# Autodesk Inventor assembly: 足裏_1_1
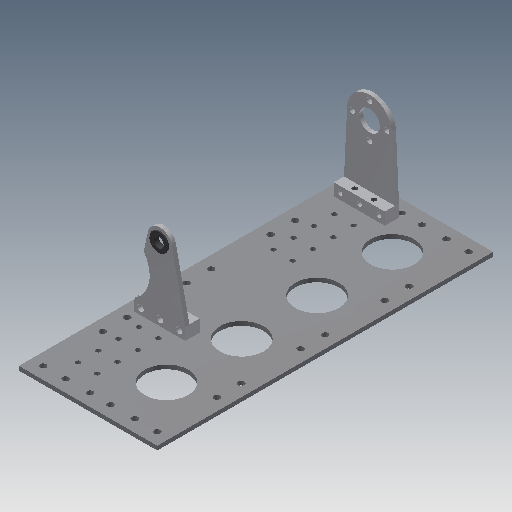
[picture p0: Inventor's stored thumbnail of the model, 512x512]
Saved by Autodesk Inventor 2017.3 (Build 213256000, 256)
## iProperties
Created: 2016-05-01
Part Number: 足裏_1_1
Document SubType Name: Assembly
Designer: hiroaki
Mass: 45.3916 g
Surface Area: 270.384 cm^2
Volume: 23.3732 cm^3
Density: 1.94204 g/cm^3
Author: hiroaki
## Documents named in this file (6)
- C:\Users\haya\Desktop\GankenKun0_5\下半身\足裏\足裏_1_1.iam
- C:\Users\haya\Desktop\GankenKun0_5\下半身\足裏\足裏_メインフレーム_1_1.ipt
- C:\Users\haya\Desktop\GankenKun0_5\下半身\足裏\足裏_メインフレーム_1_2.ipt
- C:\Users\haya\Desktop\GankenKun0_5\下半身\足裏\足裏_サブフレーム_1_1.ipt
- C:\Users\haya\Desktop\GankenKun0_5\既製品\NSK_RB_MF85ZZ\MF85ZZ.iam
- C:\Users\haya\Desktop\GankenKun0_5\下半身\足裏\足裏_メインフレーム_1_3.ipt
## Components (6 placed, 5 different names)
1. 足裏_メインフレーム_1_1:1 — メイト:1, フラッシュ:1, フラッシュ:2, メイト:2, フラッシュ:3, メイト:3, 挿入:4, 挿入:5, 挿入:6
2. 足裏_メインフレーム_1_2:1 — メイト:2, フラッシュ:3, メイト:3, 挿入:1, 挿入:2, 挿入:3, 挿入:7
3. 足裏_サブフレーム_1_1:1 — 挿入:1, 挿入:2, 挿入:3, 挿入:10, 挿入:11
4. 足裏_サブフレーム_1_1:2 — 挿入:4, 挿入:5, 挿入:6, 挿入:8, 挿入:9
5. MF85ZZ:1 [sub-assembly] — 挿入:7
6. 足裏_メインフレーム_1_3:1 — 挿入:8, 挿入:9, 挿入:10, 挿入:11
## Relationships (17: Insert 11, Mate 3, Flush 3)
- メイト:1 [Mate]: 足裏_メインフレーム_1_1:1
- フラッシュ:1 [Flush]: 足裏_メインフレーム_1_1:1
- フラッシュ:2 [Flush] (50.5 mm): 足裏_メインフレーム_1_1:1
- メイト:2 [Mate]: 足裏_メインフレーム_1_1:1 ↔ 足裏_メインフレーム_1_2:1
- フラッシュ:3 [Flush]: 足裏_メインフレーム_1_1:1 ↔ 足裏_メインフレーム_1_2:1
- メイト:3 [Mate] (101 mm): 足裏_メインフレーム_1_1:1 ↔ 足裏_メインフレーム_1_2:1
- 挿入:1 [Insert]: 足裏_メインフレーム_1_2:1 ↔ 足裏_サブフレーム_1_1:1
- 挿入:2 [Insert]: 足裏_メインフレーム_1_2:1 ↔ 足裏_サブフレーム_1_1:1
- 挿入:3 [Insert]: 足裏_メインフレーム_1_2:1 ↔ 足裏_サブフレーム_1_1:1
- 挿入:4 [Insert]: 足裏_メインフレーム_1_1:1 ↔ 足裏_サブフレーム_1_1:2
- 挿入:5 [Insert]: 足裏_メインフレーム_1_1:1 ↔ 足裏_サブフレーム_1_1:2
- 挿入:6 [Insert]: 足裏_メインフレーム_1_1:1 ↔ 足裏_サブフレーム_1_1:2
- 挿入:7 [Insert]: 足裏_メインフレーム_1_2:1 ↔ MF85ZZ:1
- 挿入:8 [Insert]: 足裏_サブフレーム_1_1:2 ↔ 足裏_メインフレーム_1_3:1
- 挿入:9 [Insert]: 足裏_サブフレーム_1_1:2 ↔ 足裏_メインフレーム_1_3:1
- 挿入:10 [Insert]: 足裏_サブフレーム_1_1:1 ↔ 足裏_メインフレーム_1_3:1
- 挿入:11 [Insert]: 足裏_サブフレーム_1_1:1 ↔ 足裏_メインフレーム_1_3:1
